# Autodesk Inventor assembly: connectorHexAssemblyForFork
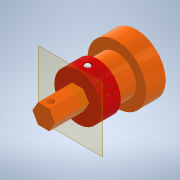
[picture p0: Inventor's stored thumbnail of the model, 180x180]
Saved by Autodesk Inventor 2022.1 (Build 261234000, 234)
## iProperties
Created: 2021-07-23
Part Number: connectorHexAssemblyForFork
Document SubType Name: Assembly
Designer: robst
Author: robst
## Documents named in this file (4)
- C:\git\CAD-Development\robSteele\ShapeWays\TelescopeProjects\TelescopeMountNov2020\connectorHexAssemblyForFork.iam
- C:\git\CAD-Development\robSteele\ShapeWays\TelescopeProjects\TelescopeMountNov2020\hexBushingForConnectorPiece.ipt
- C:\git\CAD-Development\robSteele\ShapeWays\TelescopeProjects\TelescopeMountNov2020\1_2x1_2-hexBearing.ipt
- c:\git\CAD-MfgResources\McMaster-Carr\Button Screw\6-32\6-32 x 1_125 92949A816_18-8 Stainless Steel Button Head Hex Drive Screw.ipt
## Components (3 placed, 3 different names)
1. hexBushingForConnectorPiece:1 — Insert:1
2. 1_2x1_2-hexBearing:1 — Insert:1
3. 6-32 x 1_125 92949A816_18-8 Stainless Steel Button Head Hex Drive Screw:1
## Relationships (2: Insert 2)
- Insert:1: hexBushingForConnectorPiece:1 ↔ 1_2x1_2-hexBearing:1
- [Insert]: 1_2x1_2-hexBearing:1 ↔ 6-32 x 1_125 92949A816_18-8 Stainless Steel Button Head Hex Drive Screw:1
